# Autodesk Inventor assembly: PWTR-0087
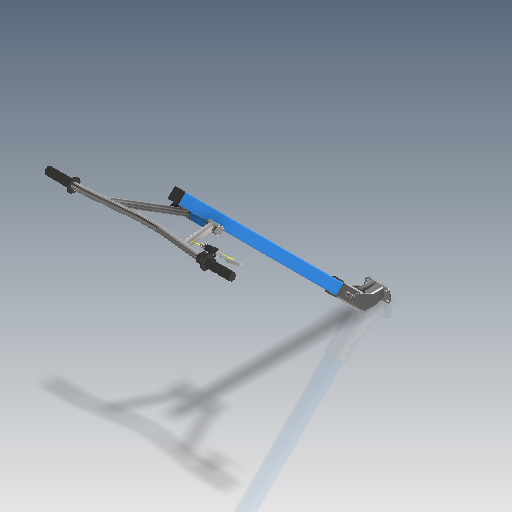
[picture p0: Inventor's stored thumbnail of the model, 512x512]
Saved by Autodesk Inventor 2021.1 (Build 251245000, 245)
## iProperties
Created: 2020-08-28
Part Number: PWTR-0087
Document SubType Name: Assembly
Designer: alid
Description: Heavy Duty Arm
Author: alid
Revision Number: A
## Documents named in this file (16)
- C:\Vault Workspace\Design Data\Projects\PRJ0095\PWTR-CTO\PWTR-0087.iam
- C:\Vault Workspace\Design Data\Projects\PRJ0095\PWTR-CTO\PWTR-0085.ipt
- C:\Vault Workspace\Design Data\Projects\PRJ0095\PWTR-CTO\PWTR-0086.ipt
- C:\Vault Workspace\Design Data\Projects\PRJ0095\PWTR-CTO\PWTR-0088.ipt
- C:\Vault Workspace\Design Data\Projects\PRJ0095\PWTR-CTO\PWTR-0089.ipt
- C:\Vault Workspace\Design Data\Projects\PRJ0095\PWTR-CTO\PWTR-0098.ipt
- C:\Vault Workspace\Design Data\Projects\PRJ0095\PWTR-CTO\PWTR-0101.ipt
- C:\Vault Workspace\Design Data\Projects\PRJ0095\PWTR-CTO\PWTR-0102.ipt
- C:\Vault Workspace\Design Data\Projects\PRJ0095\PWTR-CTO\PWTR-Supplier\PWTR-Controls\PWTR-0103.iam
- C:\Vault Workspace\Design Data\Projects\PRJ0095\PWTR-CTO\PWTR-0111.ipt
- C:\Vault Workspace\Design Data\Projects\PRJ0095\PWTR-CTO\PWTR-0112.ipt
- C:\Vault Workspace\Design Data\Projects\PRJ0095\PWTR-CTO\PWTR-0113.ipt
- C:\Vault Workspace\Design Data\Projects\PRJ0095\PWTR-CTO\PWTR-0117.ipt
- C:\Vault Workspace\Design Data\Projects\PRJ0095\PWTR-CTO\PWTR-0118.ipt
- C:\Vault Workspace\Design Data\Projects\PRJ0095\PWTR-CTO\PWTR-0122.iam
- C:\Vault Workspace\Design Data\Projects\PRJ0095\PWTR-CTO\PWTR-0123.ipt
## Components (18 placed, 16 different names)
1. HandleConn — Rigid:2, Rigid:3
2. PWTR-0086:1 — Rigid:2, Rigid:4
3. PWTR-0088:1 — Rigid:3, Rigid:5, Insert:9
4. PWTR-0089:1 — Rigid:5
5. PWTR-0089:2 — Rigid:4
6. PWTR-0103:1 [sub-assembly] — Angle:1, Mate:5
7. Bars — Angle:1, Mate:5, Insert:3, Insert:4, Insert:5
8. PWTR-0101:1 — Insert:2
9. Arm — Rigid:7
10. PWTR-0111:1 — Insert:2
11. Grip — Insert:3
12. PWTR-0112:2 — Insert:4
13. PWTR-0113:1 — Insert:5, Insert:6
14. PWTR-0117:1 — Insert:6, Insert:7, Angle:2
15. PWTR-0118:1 — Insert:7, Angle:2
16. PWTR-0122:1 [sub-assembly]
17. PWTR-0122:2 [sub-assembly] — Insert:9
18. PWTR-0123:1 — Rigid:7
## Relationships (22: Insert 9, WeldJoint 6, Mate 5, Angle 2)
- Rigid:2 [WeldJoint]: HandleConn ↔ PWTR-0086:1
- Rigid:3 [WeldJoint]: HandleConn ↔ PWTR-0088:1
- Rigid:4 [WeldJoint]: PWTR-0086:1 ↔ PWTR-0089:2
- Rigid:5 [WeldJoint]: PWTR-0088:1 ↔ PWTR-0089:1
- [Mate]: PWTR-0088:1 ↔ Arm
- [Mate]: PWTR-0088:1 ↔ Arm
- [WeldJoint]: PWTR-0101:1 ↔ Arm
- [Insert]: Bars ↔ Arm
- [Mate]: PWTR-0088:1 ↔ Arm
- [Mate]: PWTR-0103:1 ↔ Bars
- Insert:2: PWTR-0101:1 ↔ PWTR-0111:1
- Angle:1 (160 deg): PWTR-0103:1 ↔ Bars
- Mate:5: PWTR-0103:1 ↔ Bars
- Insert:3: Bars ↔ Grip
- Insert:4: Bars ↔ PWTR-0112:2
- Insert:5: Bars ↔ PWTR-0113:1
- Insert:6: PWTR-0113:1 ↔ PWTR-0117:1
- Insert:7: PWTR-0117:1 ↔ PWTR-0118:1
- Angle:2 (0 deg): PWTR-0117:1 ↔ PWTR-0118:1
- [Insert]: PWTR-0088:1 ↔ PWTR-0122:1
- Insert:9: PWTR-0088:1 ↔ PWTR-0122:2
- Rigid:7 [WeldJoint]: Arm ↔ PWTR-0123:1
